# Autodesk Inventor assembly: 足裏_1_1_MIR
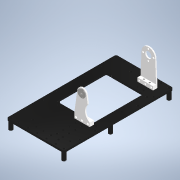
[picture p0: Inventor's stored thumbnail of the model, 180x180]
Saved by Autodesk Inventor 2020.3 (Build 243373000, 373)
## iProperties
Created: 2016-05-01
Part Number: 足裏_1_1_MIR
Document SubType Name: Assembly
Designer: masato
Mass: 45.5975 g
Surface Area: 270.055 cm^2
Volume: 23.2522 cm^3
Density: 1.96099 g/cm^3
Author: hiroaki
## Documents named in this file (7)
- C:\Users\masato\Documents\Inventor\CITBrains\スパイク\OpenPlatform_ver3_0\下半身\足裏\足裏_1_1_MIR.iam
- C:\Users\masato\Documents\Inventor\CITBrains\スパイク\OpenPlatform_ver3_0\下半身\足裏\足裏_メインフレーム_1_1.ipt
- C:\Users\masato\Documents\Inventor\CITBrains\スパイク\OpenPlatform_ver3_0\下半身\足裏\足裏_メインフレーム_1_2.ipt
- C:\Users\masato\Documents\Inventor\CITBrains\スパイク\OpenPlatform_ver3_0\下半身\足裏\足裏_サブフレーム_1_1.ipt
- C:\Users\masato\Documents\Inventor\CITBrains\スパイク\OpenPlatform_ver3_0\既製品\NSK_RB_F694ZZ\F694ZZ.iam
- C:\Users\masato\Documents\Inventor\CITBrains\スパイク\OpenPlatform_ver3_0\下半身\足裏\足裏_メインフレーム_2_3.ipt
- C:\Users\masato\Documents\Inventor\CITBrains\スパイク\OpenPlatform_ver3_0\既製品\ARL-313SBE.ipt
## Components (12 placed, 6 different names)
1. 足裏_メインフレーム_1_1:1 — フラッシュ:2, フラッシュ:1, メイト:1, フラッシュ:3, メイト:2, 挿入:6, 挿入:5, 挿入:4
2. 足裏_メインフレーム_1_2:1 — フラッシュ:3, メイト:2, 挿入:3, 挿入:2, 挿入:1, 挿入:12
3. 足裏_サブフレーム_1_1:1 — 挿入:3, 挿入:2, 挿入:1, 挿入:16, 挿入:15
4. 足裏_サブフレーム_1_1:2 — 挿入:6, 挿入:5, 挿入:4, 挿入:14, 挿入:13
5. F694ZZ:1 [sub-assembly] — 挿入:12
6. 足裏_メインフレーム_2_3:1 — 挿入:16, 挿入:15, 挿入:14, 挿入:13, 挿入:17, 挿入:18, 挿入:19, 挿入:20, 挿入:22, 挿入:21
7. ARL-313SBE:1 — 挿入:17
8. ARL-313SBE:2 — 挿入:18
9. ARL-313SBE:3 — 挿入:19
10. ARL-313SBE:4 — 挿入:20
11. ARL-313SBE:5 — 挿入:22
12. ARL-313SBE:6 — 挿入:21
## Relationships (22: Insert 17, Flush 3, Mate 2)
- フラッシュ:2 [Flush] (50.5 mm): 足裏_メインフレーム_1_1:1
- フラッシュ:1 [Flush]: 足裏_メインフレーム_1_1:1
- メイト:1 [Mate]: 足裏_メインフレーム_1_1:1
- フラッシュ:3 [Flush]: 足裏_メインフレーム_1_1:1 ↔ 足裏_メインフレーム_1_2:1
- メイト:2 [Mate]: 足裏_メインフレーム_1_1:1 ↔ 足裏_メインフレーム_1_2:1
- 挿入:3 [Insert]: 足裏_メインフレーム_1_2:1 ↔ 足裏_サブフレーム_1_1:1
- 挿入:2 [Insert]: 足裏_メインフレーム_1_2:1 ↔ 足裏_サブフレーム_1_1:1
- 挿入:1 [Insert]: 足裏_メインフレーム_1_2:1 ↔ 足裏_サブフレーム_1_1:1
- 挿入:6 [Insert]: 足裏_メインフレーム_1_1:1 ↔ 足裏_サブフレーム_1_1:2
- 挿入:5 [Insert]: 足裏_メインフレーム_1_1:1 ↔ 足裏_サブフレーム_1_1:2
- 挿入:4 [Insert]: 足裏_メインフレーム_1_1:1 ↔ 足裏_サブフレーム_1_1:2
- 挿入:12 [Insert]: 足裏_メインフレーム_1_2:1 ↔ F694ZZ:1
- 挿入:16 [Insert]: 足裏_サブフレーム_1_1:1 ↔ 足裏_メインフレーム_2_3:1
- 挿入:15 [Insert]: 足裏_サブフレーム_1_1:1 ↔ 足裏_メインフレーム_2_3:1
- 挿入:14 [Insert]: 足裏_サブフレーム_1_1:2 ↔ 足裏_メインフレーム_2_3:1
- 挿入:13 [Insert]: 足裏_サブフレーム_1_1:2 ↔ 足裏_メインフレーム_2_3:1
- 挿入:17 [Insert]: 足裏_メインフレーム_2_3:1 ↔ ARL-313SBE:1
- 挿入:18 [Insert]: 足裏_メインフレーム_2_3:1 ↔ ARL-313SBE:2
- 挿入:19 [Insert]: 足裏_メインフレーム_2_3:1 ↔ ARL-313SBE:3
- 挿入:20 [Insert]: 足裏_メインフレーム_2_3:1 ↔ ARL-313SBE:4
- 挿入:22 [Insert]: 足裏_メインフレーム_2_3:1 ↔ ARL-313SBE:5
- 挿入:21 [Insert]: 足裏_メインフレーム_2_3:1 ↔ ARL-313SBE:6
